# Autodesk Inventor assembly: Catapult Launcher
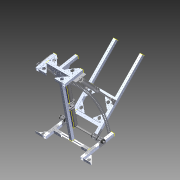
[picture p0: Inventor's stored thumbnail of the model, 180x180]
Saved by Autodesk Inventor 2014 (Build 180170000, 170)
## iProperties
Created: 2014-01-17
Part Number: Catapult Launcher
Document SubType Name: Assembly
Designer: Andrew Toennies
Mass: 5501.43 g
Surface Area: 13469.8 cm^2
Volume: 1150.51 cm^3
Density: 4.78173 g/cm^3
Author: Andrew Toennies
## Documents named in this file (26)
- C:\Users\Michael\Documents\GitHub\2014buildCAD\New Shooter\Catapult Launcher.iam
- C:\Users\Michael\Documents\GitHub\2014buildCAD\New Shooter\Vex Pro 1x1 rectangular tubing 7 in length.ipt
- C:\Users\Michael\Documents\GitHub\2014buildCAD\New Shooter\Vex Pro Side Bearing Gusset - OUT OF STOCK 1192014.ipt
- C:\Users\Michael\Documents\GitHub\2014buildCAD\New Shooter\Vex Pro Corner Gusset - IN STOCK 1192014.ipt
- C:\Users\Michael\Documents\GitHub\2014buildCAD\New Shooter\Bearing ID 0.500 Hex OD 1.125.ipt
- C:\Users\Michael\Documents\GitHub\2014buildCAD\New Shooter\Shaft (Steel 0.500 Hex).ipt
- C:\Users\Michael\Documents\GitHub\2014buildCAD\New Shooter\Vex Pro 1x1 rectangular tubing 27 in length.ipt
- C:\Users\Michael\Documents\GitHub\2014buildCAD\New Shooter\Vex Pro 1x1 rectangular tubing 3 in length.ipt
- C:\Users\Michael\Documents\GitHub\2014buildCAD\New Shooter\Vex Pro 1x1 rectangular tubing 11 in length.ipt
- C:\Users\Michael\Documents\GitHub\2014buildCAD\New Shooter\1.5 in bore 6 in stroke cylinder - BIMBA\176-DP(D-229)(F,D-231-1).iam
- C:\Users\Michael\Documents\GitHub\2014buildCAD\New Shooter\Aluminum Plate (0.125).ipt
- C:\Users\Michael\Documents\GitHub\2014buildCAD\New Shooter\1.5 in bore 6 in stroke cylinder - BIMBA\D-14826.ipt
- C:\Users\Michael\Documents\GitHub\2014buildCAD\New Shooter\1.5 in bore 6 in stroke cylinder - BIMBA\D-9969.ipt
- C:\Users\Michael\Documents\GitHub\2014buildCAD\New Shooter\Vex Pro End Bearing Mount - IN STOCK 1192014.ipt
- C:\Users\Michael\Documents\GitHub\2014buildCAD\New Shooter\Vex Pro 1x1 rectangular tubing 13 in length.ipt
- C:\Users\Michael\Documents\GitHub\2014buildCAD\New Shooter\Vex Pro 1x1 rectangular tubing 25 in length.ipt
- C:\Users\Michael\Documents\GitHub\2014buildCAD\New Shooter\0.5625 in bore 2 in stroke compact cylinder - BIMBA\FO-022.iam
- C:\Users\Michael\Documents\GitHub\2014buildCAD\New Shooter\Vex Pro 1x1 rectangular tubing 8 in length.ipt
- C:\Users\Michael\Documents\GitHub\2014buildCAD\New Shooter\Hex Shaft Collar 1-2 in (7552K500).ipt
- C:\Users\Michael\Documents\GitHub\2014buildCAD\New Shooter\#8 1 in length standoff 93330A459.ipt
- C:\Users\Michael\Documents\GitHub\2014buildCAD\New Shooter\Ramp.ipt
- C:\Users\Michael\Documents\GitHub\2014buildCAD\New folder (2)\Pneumatics_Clippard_AVT-32-16.iam
- C:\Users\Michael\Documents\GitHub\2014buildCAD\New Shooter\Spacer (0.4375 ID whatever OD) aluminum.ipt
- C:\Users\Michael\Documents\GitHub\2014buildCAD\New Shooter\Vex Pro T gusset - OUT OF STOCK 1192014.ipt
- C:\Users\Michael\Documents\GitHub\2014buildCAD\New Shooter\#8 0.250 in length spacer 92510A462.ipt
- C:\Users\Michael\Documents\GitHub\2014buildCAD\New Shooter\#8 0.625 in length spacer 92510A466.ipt
## Components (84 placed, 25 different names)
1. Vex Pro T gusset - OUT OF STOCK 1192014:3 — Mate:388, Flush:73, Flush:74
2. Vex Pro T gusset - OUT OF STOCK 1192014:2 — Mate:376, Flush:71, Flush:72
3. Vex Pro T gusset - OUT OF STOCK 1192014:1 — Mate:375, Flush:69, Flush:70
4. #8 1 in length standoff 93330A459:12 — Mate:342, Mate:343
5. #8 1 in length standoff 93330A459:11 — Mate:340, Mate:341
6. #8 1 in length standoff 93330A459:10 — Mate:338, Mate:339
7. #8 1 in length standoff 93330A459:9 — Mate:336, Mate:337
8. #8 1 in length standoff 93330A459:6 — Mate:325, Mate:326
9. #8 1 in length standoff 93330A459:1 — Mate:319, Mate:320
10. #8 1 in length standoff 93330A459:2 — Mate:321, Mate:322
11. #8 1 in length standoff 93330A459:5 — Mate:323, Mate:324
12. Vex Pro 1x1 rectangular tubing 7 in length:1 — Flush:1, Flush:2, Mate:8, Mate:11, Mate:23, Mate:24, Mate:25, Mate:195, Flush:32, Flush:33, Flush:34, Flush:35, Mate:278, Flush:51, Mate:352, Mate:376, Flush:71, Mate:380, Mate:381
13. Vex Pro 1x1 rectangular tubing 7 in length:2 — Flush:1, Flush:2, Mate:3, Mate:5, Mate:14, Mate:15, Mate:16, Mate:123, Mate:188, Mate:195, Flush:25, Flush:28, Flush:29, Flush:30, Flush:31, Mate:355, Mate:375, Flush:69, Mate:378
14. Vex Pro Side Bearing Gusset - OUT OF STOCK 1192014:1 — Mate:3, Mate:26, Mate:27, Flush:28, Flush:29, Mate:319, Mate:320, Mate:322, Mate:324, Mate:326
15. Vex Pro Side Bearing Gusset - OUT OF STOCK 1192014:2 — Mate:5, Mate:28, Mate:29, Flush:30, Flush:31, Mate:321, Mate:323, Mate:325
16. Vex Pro Side Bearing Gusset - OUT OF STOCK 1192014:3 — Mate:11, Mate:32, Mate:33, Flush:32, Flush:33, Mate:337, Mate:338, Mate:339, Mate:340, Mate:342, Mate:343
17. Vex Pro Side Bearing Gusset - OUT OF STOCK 1192014:4 — Mate:8, Mate:30, Mate:31, Flush:34, Flush:35, Mate:336, Mate:341
18. Vex Pro Corner Gusset - IN STOCK 1192014:2 — Mate:14, Mate:15, Mate:16, Flush:53
19. Vex Pro Corner Gusset - IN STOCK 1192014:4 — Mate:23, Mate:24, Mate:25
20. Bearing ID 0.500 Hex OD 1.125:1 — Mate:28, Mate:29, Flush:3, Flush:5, Mate:306
21. Bearing ID 0.500 Hex OD 1.125:2 — Mate:26, Mate:27, Flush:3, Mate:34, Mate:35, Mate:303
22. Bearing ID 0.500 Hex OD 1.125:3 — Mate:30, Mate:31, Flush:4, Mate:318
23. Bearing ID 0.500 Hex OD 1.125:4 — Mate:32, Mate:33, Flush:4, Flush:5, Mate:69, Mate:315
24. Spacer (0.4375 ID whatever OD) aluminum:1 — Mate:371, Mate:372
25. Spacer (0.4375 ID whatever OD) aluminum:2 — Mate:373, Mate:374
26. Shaft (Steel 0.500 Hex):1 — Mate:34, Mate:35, Flush:25, Mate:227, Mate:228, Mate:301, Mate:302, Mate:304, Mate:305, Mate:307, Mate:308, Mate:310, Mate:311, Mate:313, Mate:314, Mate:316, Mate:317
27. Hex Shaft Collar 1-2 in (7552K500):1 — Mate:301, Mate:302, Mate:303
28. Hex Shaft Collar 1-2 in (7552K500):2 — Mate:307, Mate:308, Mate:309
29. Hex Shaft Collar 1-2 in (7552K500):3 — Mate:304, Mate:305, Mate:306, Mate:371, Mate:372
30. Hex Shaft Collar 1-2 in (7552K500):4 — Mate:310, Mate:311, Mate:312
31. Hex Shaft Collar 1-2 in (7552K500):5 — Mate:313, Mate:314, Mate:315, Mate:373, Mate:374
32. Hex Shaft Collar 1-2 in (7552K500):6 — Mate:316, Mate:317, Mate:318
33. #8 1 in length standoff 93330A459:13 — Mate:350, Mate:351
34. #8 1 in length standoff 93330A459:14 — Mate:348, Mate:349
35. #8 1 in length standoff 93330A459:15 — Mate:346, Mate:347
36. #8 1 in length standoff 93330A459:16 — Mate:344, Mate:345
37. #8 1 in length standoff 93330A459:3 — Mate:327, Mate:328
38. #8 1 in length standoff 93330A459:4 — Mate:329, Mate:330
39. #8 1 in length standoff 93330A459:7 — Mate:334, Mate:335
40. #8 1 in length standoff 93330A459:8 — Mate:332, Mate:333
41. Vex Pro Corner Gusset - IN STOCK 1192014:14 — Mate:250, Mate:251, Flush:45, Mate:271
42. Vex Pro Corner Gusset - IN STOCK 1192014:13 — Mate:252, Mate:253, Flush:46
43. Vex Pro Corner Gusset - IN STOCK 1192014:12 — Mate:248, Mate:249, Flush:44
44. Vex Pro Corner Gusset - IN STOCK 1192014:11 — Mate:243, Flush:43, Mate:244
45. Vex Pro 1x1 rectangular tubing 11 in length:1 — Mate:191, Flush:42, Mate:250, Mate:253, Flush:46, Mate:267
46. Vex Pro 1x1 rectangular tubing 11 in length:2 — Flush:41, Mate:242, Mate:243, Flush:43, Mate:246, Mate:248, Flush:44
47. D-9969:1 — Mate:164, Mate:165, Mate:198, Flush:36, Mate:270, Mate:377
48. D-14826:1 — Mate:164, Mate:169, Mate:170, Flush:37, Mate:247
49. Vex Pro End Bearing Mount - IN STOCK 1192014:4 — Mate:229, Mate:230, Mate:231, Mate:232, Mate:246, Mate:345, Mate:346, Mate:348, Mate:349, Mate:350
50. Vex Pro End Bearing Mount - IN STOCK 1192014:3 — Mate:217, Mate:218, Mate:219, Mate:220, Mate:221, Mate:327, Mate:328, Mate:330, Mate:333, Mate:335
51. Vex Pro End Bearing Mount - IN STOCK 1192014:2 — Mate:233, Mate:234, Mate:235, Mate:236, Mate:245, Mate:344, Mate:347, Mate:351
52. Vex Pro End Bearing Mount - IN STOCK 1192014:1 — Mate:222, Mate:223, Mate:224, Mate:225, Mate:226, Mate:329, Mate:332, Mate:334
53. Vex Pro 1x1 rectangular tubing 27 in length:3 — Mate:198, Mate:229, Mate:230, Mate:231, Mate:233, Mate:234, Mate:235, Flush:27, Flush:36, Flush:41, Mate:242, Mate:244, Mate:251, Flush:45, Mate:267, Mate:270, Mate:271
54. Vex Pro 1x1 rectangular tubing 27 in length:2 — Mate:188, Mate:191, Mate:212, Mate:219, Mate:220, Mate:221, Mate:224, Mate:225, Mate:226, Flush:26, Flush:37, Flush:42, Mate:247, Mate:249, Mate:252
55. Bearing ID 0.500 Hex OD 1.125:5 — Mate:80, Mate:222, Mate:223, Mate:228, Mate:309
56. Bearing ID 0.500 Hex OD 1.125:6 — Mate:80, Mate:217, Mate:218, Mate:227
57. Bearing ID 0.500 Hex OD 1.125:7 — Mate:68, Mate:69, Mate:236, Mate:245
58. Bearing ID 0.500 Hex OD 1.125:8 — Mate:68, Mate:232, Mate:312
59. 176-DP(D-229)(F,D-231-1):1 [sub-assembly] — Mate:153, Mate:154, Mate:155, Mate:165, Mate:171, Mate:377
60. 176-DP(D-229)(F,D-231-1):2 [sub-assembly] — Mate:156, Mate:167, Mate:168, Mate:169, Mate:170, Mate:171
61. Aluminum Plate (0.125):1 — Mate:153, Mate:154, Mate:155, Mate:159, Flush:24
62. Aluminum Plate (0.125):2 — Mate:156, Mate:160, Mate:167, Mate:168, Flush:24, Flush:47
63. Vex Pro 1x1 rectangular tubing 3 in length:2 — Mate:121, Flush:14, Mate:122, Flush:19, Mate:159, Flush:27, Mate:276, Mate:359, Mate:385
64. Vex Pro 1x1 rectangular tubing 3 in length:1 — Flush:13, Mate:118, Mate:119, Mate:120, Mate:123, Flush:19, Mate:160, Mate:212, Flush:26, Flush:47, Mate:272, Flush:48, Mate:273, Mate:275, Mate:360, Mate:387
65. Vex Pro Corner Gusset - IN STOCK 1192014:8 — Flush:13, Mate:118, Mate:119, Mate:120, Flush:17, Flush:53
66. Vex Pro Corner Gusset - IN STOCK 1192014:6 — Mate:121, Flush:14, Mate:122, Flush:17
67. Vex Pro 1x1 rectangular tubing 11 in length:3 — Mate:272, Flush:48, Mate:274, Flush:49, Mate:277, Flush:50, Mate:290, Mate:291, Mate:293, Flush:57, Mate:369, Flush:66
68. Vex Pro Corner Gusset - IN STOCK 1192014:15 — Mate:273, Mate:274, Flush:49, Mate:275
69. Vex Pro Corner Gusset - IN STOCK 1192014:16 — Mate:276, Mate:277, Flush:50
70. Vex Pro 1x1 rectangular tubing 13 in length:1 — Mate:278, Flush:51, Mate:284, Flush:55, Flush:65, Flush:70, Flush:72, Mate:388, Flush:73
71. Vex Pro 1x1 rectangular tubing 25 in length:1 — Mate:284, Flush:55, Mate:285, Mate:287, Mate:288, Mate:289, Flush:56, Mate:292, Mate:300, Flush:63, Mate:367, Flush:64, Mate:368, Flush:67, Flush:74
72. FO-022:1 [sub-assembly] — Mate:285, Mate:287, Mate:288
73. Vex Pro Corner Gusset - IN STOCK 1192014:17 — Mate:289, Mate:290, Flush:56, Mate:291
74. Vex Pro Corner Gusset - IN STOCK 1192014:18 — Mate:292, Mate:293, Flush:57
75. Vex Pro 1x1 rectangular tubing 8 in length:1 — Mate:369, Flush:66, Mate:370, Flush:68
76. Vex Pro Corner Gusset - IN STOCK 1192014:21 — Mate:300, Mate:370, Flush:67, Flush:68
77. #8 0.250 in length spacer 92510A462:1 — Mate:380, Mate:381, Mate:382
78. #8 0.250 in length spacer 92510A462:2 — Mate:378, Mate:379, Mate:383
79. #8 0.625 in length spacer 92510A466:1 — Mate:384, Mate:385
80. #8 0.625 in length spacer 92510A466:2 — Mate:386, Mate:387
81. Ramp:1 — Mate:355, Mate:360, Mate:379, Mate:383, Mate:386
82. Ramp:2 — Mate:352, Mate:359, Mate:382, Mate:384
83. Pneumatics_Clippard_AVT-32-16:1 [sub-assembly] — Flush:63, Mate:367, Flush:65
84. Pneumatics_Clippard_AVT-32-16:2 [sub-assembly] — Flush:64, Mate:368
## Relationships (225: Mate 175, Flush 50)
- Flush:1: Vex Pro 1x1 rectangular tubing 7 in length:1 ↔ Vex Pro 1x1 rectangular tubing 7 in length:2
- Flush:2: Vex Pro 1x1 rectangular tubing 7 in length:1 ↔ Vex Pro 1x1 rectangular tubing 7 in length:2
- Mate:3: Vex Pro 1x1 rectangular tubing 7 in length:2 ↔ Vex Pro Side Bearing Gusset - OUT OF STOCK 1192014:1
- Mate:5: Vex Pro 1x1 rectangular tubing 7 in length:2 ↔ Vex Pro Side Bearing Gusset - OUT OF STOCK 1192014:2
- Mate:8: Vex Pro 1x1 rectangular tubing 7 in length:1 ↔ Vex Pro Side Bearing Gusset - OUT OF STOCK 1192014:4
- Mate:11: Vex Pro 1x1 rectangular tubing 7 in length:1 ↔ Vex Pro Side Bearing Gusset - OUT OF STOCK 1192014:3
- Mate:14: Vex Pro 1x1 rectangular tubing 7 in length:2 ↔ Vex Pro Corner Gusset - IN STOCK 1192014:2
- Mate:15: Vex Pro 1x1 rectangular tubing 7 in length:2 ↔ Vex Pro Corner Gusset - IN STOCK 1192014:2
- Mate:16: Vex Pro 1x1 rectangular tubing 7 in length:2 ↔ Vex Pro Corner Gusset - IN STOCK 1192014:2
- Mate:23: Vex Pro 1x1 rectangular tubing 7 in length:1 ↔ Vex Pro Corner Gusset - IN STOCK 1192014:4
- Mate:24: Vex Pro 1x1 rectangular tubing 7 in length:1 ↔ Vex Pro Corner Gusset - IN STOCK 1192014:4
- Mate:25: Vex Pro 1x1 rectangular tubing 7 in length:1 ↔ Vex Pro Corner Gusset - IN STOCK 1192014:4
- Mate:26: Vex Pro Side Bearing Gusset - OUT OF STOCK 1192014:1 ↔ Bearing ID 0.500 Hex OD 1.125:2
- Mate:27: Vex Pro Side Bearing Gusset - OUT OF STOCK 1192014:1 ↔ Bearing ID 0.500 Hex OD 1.125:2
- Mate:28: Vex Pro Side Bearing Gusset - OUT OF STOCK 1192014:2 ↔ Bearing ID 0.500 Hex OD 1.125:1
- Mate:29: Vex Pro Side Bearing Gusset - OUT OF STOCK 1192014:2 ↔ Bearing ID 0.500 Hex OD 1.125:1
- Flush:3: Bearing ID 0.500 Hex OD 1.125:1 ↔ Bearing ID 0.500 Hex OD 1.125:2
- Mate:30: Vex Pro Side Bearing Gusset - OUT OF STOCK 1192014:4 ↔ Bearing ID 0.500 Hex OD 1.125:3
- Mate:31: Vex Pro Side Bearing Gusset - OUT OF STOCK 1192014:4 ↔ Bearing ID 0.500 Hex OD 1.125:3
- Mate:32: Vex Pro Side Bearing Gusset - OUT OF STOCK 1192014:3 ↔ Bearing ID 0.500 Hex OD 1.125:4
- Mate:33: Vex Pro Side Bearing Gusset - OUT OF STOCK 1192014:3 ↔ Bearing ID 0.500 Hex OD 1.125:4
- Flush:4: Bearing ID 0.500 Hex OD 1.125:3 ↔ Bearing ID 0.500 Hex OD 1.125:4
- Flush:5: Bearing ID 0.500 Hex OD 1.125:1 ↔ Bearing ID 0.500 Hex OD 1.125:4
- Mate:34: Bearing ID 0.500 Hex OD 1.125:2 ↔ Shaft (Steel 0.500 Hex):1
- Mate:35: Bearing ID 0.500 Hex OD 1.125:2 ↔ Shaft (Steel 0.500 Hex):1
- Mate:68: Bearing ID 0.500 Hex OD 1.125:7 ↔ Bearing ID 0.500 Hex OD 1.125:8
- Mate:69: Bearing ID 0.500 Hex OD 1.125:4 ↔ Bearing ID 0.500 Hex OD 1.125:7
- Mate:80: Bearing ID 0.500 Hex OD 1.125:5 ↔ Bearing ID 0.500 Hex OD 1.125:6
- Flush:13: Vex Pro 1x1 rectangular tubing 3 in length:1 ↔ Vex Pro Corner Gusset - IN STOCK 1192014:8
- Mate:118: Vex Pro 1x1 rectangular tubing 3 in length:1 ↔ Vex Pro Corner Gusset - IN STOCK 1192014:8
- Mate:119: Vex Pro 1x1 rectangular tubing 3 in length:1 ↔ Vex Pro Corner Gusset - IN STOCK 1192014:8
- Mate:120: Vex Pro 1x1 rectangular tubing 3 in length:1 ↔ Vex Pro Corner Gusset - IN STOCK 1192014:8
- Mate:121: Vex Pro 1x1 rectangular tubing 3 in length:2 ↔ Vex Pro Corner Gusset - IN STOCK 1192014:6
- Flush:14: Vex Pro 1x1 rectangular tubing 3 in length:2 ↔ Vex Pro Corner Gusset - IN STOCK 1192014:6
- Mate:122: Vex Pro 1x1 rectangular tubing 3 in length:2 ↔ Vex Pro Corner Gusset - IN STOCK 1192014:6
- Flush:17: Vex Pro Corner Gusset - IN STOCK 1192014:8 ↔ Vex Pro Corner Gusset - IN STOCK 1192014:6
- Mate:123 (-685.8 mm): Vex Pro 1x1 rectangular tubing 7 in length:2 ↔ Vex Pro 1x1 rectangular tubing 3 in length:1
- Flush:19: Vex Pro 1x1 rectangular tubing 3 in length:2 ↔ Vex Pro 1x1 rectangular tubing 3 in length:1
- Mate:153: 176-DP(D-229)(F,D-231-1):1 ↔ Aluminum Plate (0.125):1
- Mate:154: 176-DP(D-229)(F,D-231-1):1 ↔ Aluminum Plate (0.125):1
- Mate:155: 176-DP(D-229)(F,D-231-1):1 ↔ Aluminum Plate (0.125):1
- Mate:156: 176-DP(D-229)(F,D-231-1):2 ↔ Aluminum Plate (0.125):2
- Mate:159: Aluminum Plate (0.125):1 ↔ Vex Pro 1x1 rectangular tubing 3 in length:2
- Mate:160: Aluminum Plate (0.125):2 ↔ Vex Pro 1x1 rectangular tubing 3 in length:1
- Mate:164: D-9969:1 ↔ D-14826:1
- Mate:165: D-9969:1 ↔ 176-DP(D-229)(F,D-231-1):1
- Mate:167: 176-DP(D-229)(F,D-231-1):2 ↔ Aluminum Plate (0.125):2
- Mate:168: 176-DP(D-229)(F,D-231-1):2 ↔ Aluminum Plate (0.125):2
- Mate:169: D-14826:1 ↔ 176-DP(D-229)(F,D-231-1):2
- Mate:170: D-14826:1 ↔ 176-DP(D-229)(F,D-231-1):2
- Mate:171: 176-DP(D-229)(F,D-231-1):1 ↔ 176-DP(D-229)(F,D-231-1):2
- Flush:24: Aluminum Plate (0.125):1 ↔ Aluminum Plate (0.125):2
- Mate:188 (25.4 mm): Vex Pro 1x1 rectangular tubing 7 in length:2 ↔ Vex Pro 1x1 rectangular tubing 27 in length:2
- Mate:191: Vex Pro 1x1 rectangular tubing 11 in length:1 ↔ Vex Pro 1x1 rectangular tubing 27 in length:2
- Mate:195 (330.2 mm): Vex Pro 1x1 rectangular tubing 7 in length:1 ↔ Vex Pro 1x1 rectangular tubing 7 in length:2
- Flush:25 (-25.4 mm): Vex Pro 1x1 rectangular tubing 7 in length:2 ↔ Shaft (Steel 0.500 Hex):1
- Mate:198: D-9969:1 ↔ Vex Pro 1x1 rectangular tubing 27 in length:3
- Mate:212: Vex Pro 1x1 rectangular tubing 27 in length:2 ↔ Vex Pro 1x1 rectangular tubing 3 in length:1
- Mate:217: Vex Pro End Bearing Mount - IN STOCK 1192014:3 ↔ Bearing ID 0.500 Hex OD 1.125:6
- Mate:218: Vex Pro End Bearing Mount - IN STOCK 1192014:3 ↔ Bearing ID 0.500 Hex OD 1.125:6
- Mate:219: Vex Pro End Bearing Mount - IN STOCK 1192014:3 ↔ Vex Pro 1x1 rectangular tubing 27 in length:2
- Mate:220: Vex Pro End Bearing Mount - IN STOCK 1192014:3 ↔ Vex Pro 1x1 rectangular tubing 27 in length:2
- Mate:221: Vex Pro End Bearing Mount - IN STOCK 1192014:3 ↔ Vex Pro 1x1 rectangular tubing 27 in length:2
- Mate:222: Vex Pro End Bearing Mount - IN STOCK 1192014:1 ↔ Bearing ID 0.500 Hex OD 1.125:5
- Mate:223: Vex Pro End Bearing Mount - IN STOCK 1192014:1 ↔ Bearing ID 0.500 Hex OD 1.125:5
- Mate:224: Vex Pro End Bearing Mount - IN STOCK 1192014:1 ↔ Vex Pro 1x1 rectangular tubing 27 in length:2
- Mate:225: Vex Pro End Bearing Mount - IN STOCK 1192014:1 ↔ Vex Pro 1x1 rectangular tubing 27 in length:2
- Mate:226: Vex Pro End Bearing Mount - IN STOCK 1192014:1 ↔ Vex Pro 1x1 rectangular tubing 27 in length:2
- Mate:227: Shaft (Steel 0.500 Hex):1 ↔ Bearing ID 0.500 Hex OD 1.125:6
- Mate:228: Shaft (Steel 0.500 Hex):1 ↔ Bearing ID 0.500 Hex OD 1.125:5
- Mate:229: Vex Pro End Bearing Mount - IN STOCK 1192014:4 ↔ Vex Pro 1x1 rectangular tubing 27 in length:3
- Mate:230: Vex Pro End Bearing Mount - IN STOCK 1192014:4 ↔ Vex Pro 1x1 rectangular tubing 27 in length:3
- Mate:231: Vex Pro End Bearing Mount - IN STOCK 1192014:4 ↔ Vex Pro 1x1 rectangular tubing 27 in length:3
- Mate:232: Vex Pro End Bearing Mount - IN STOCK 1192014:4 ↔ Bearing ID 0.500 Hex OD 1.125:8
- Mate:233: Vex Pro End Bearing Mount - IN STOCK 1192014:2 ↔ Vex Pro 1x1 rectangular tubing 27 in length:3
- Mate:234: Vex Pro End Bearing Mount - IN STOCK 1192014:2 ↔ Vex Pro 1x1 rectangular tubing 27 in length:3
- Mate:235: Vex Pro End Bearing Mount - IN STOCK 1192014:2 ↔ Vex Pro 1x1 rectangular tubing 27 in length:3
- Mate:236: Vex Pro End Bearing Mount - IN STOCK 1192014:2 ↔ Bearing ID 0.500 Hex OD 1.125:7
- Flush:26: Vex Pro 1x1 rectangular tubing 27 in length:2 ↔ Vex Pro 1x1 rectangular tubing 3 in length:1
- Flush:27: Vex Pro 1x1 rectangular tubing 27 in length:3 ↔ Vex Pro 1x1 rectangular tubing 3 in length:2
- Flush:28: Vex Pro 1x1 rectangular tubing 7 in length:2 ↔ Vex Pro Side Bearing Gusset - OUT OF STOCK 1192014:1
- Flush:29 (82.55 mm): Vex Pro 1x1 rectangular tubing 7 in length:2 ↔ Vex Pro Side Bearing Gusset - OUT OF STOCK 1192014:1
- Flush:30: Vex Pro 1x1 rectangular tubing 7 in length:2 ↔ Vex Pro Side Bearing Gusset - OUT OF STOCK 1192014:2
- Flush:31 (-82.55 mm): Vex Pro 1x1 rectangular tubing 7 in length:2 ↔ Vex Pro Side Bearing Gusset - OUT OF STOCK 1192014:2
- Flush:32: Vex Pro 1x1 rectangular tubing 7 in length:1 ↔ Vex Pro Side Bearing Gusset - OUT OF STOCK 1192014:3
- Flush:33 (82.55 mm): Vex Pro 1x1 rectangular tubing 7 in length:1 ↔ Vex Pro Side Bearing Gusset - OUT OF STOCK 1192014:3
- Flush:34: Vex Pro 1x1 rectangular tubing 7 in length:1 ↔ Vex Pro Side Bearing Gusset - OUT OF STOCK 1192014:4
- Flush:35 (-82.55 mm): Vex Pro 1x1 rectangular tubing 7 in length:1 ↔ Vex Pro Side Bearing Gusset - OUT OF STOCK 1192014:4
- Flush:36: D-9969:1 ↔ Vex Pro 1x1 rectangular tubing 27 in length:3
- Flush:37: D-14826:1 ↔ Vex Pro 1x1 rectangular tubing 27 in length:2
- Flush:41: Vex Pro 1x1 rectangular tubing 11 in length:2 ↔ Vex Pro 1x1 rectangular tubing 27 in length:3
- Mate:242: Vex Pro 1x1 rectangular tubing 11 in length:2 ↔ Vex Pro 1x1 rectangular tubing 27 in length:3
- Flush:42: Vex Pro 1x1 rectangular tubing 11 in length:1 ↔ Vex Pro 1x1 rectangular tubing 27 in length:2
- Mate:243: Vex Pro Corner Gusset - IN STOCK 1192014:11 ↔ Vex Pro 1x1 rectangular tubing 11 in length:2
- Flush:43: Vex Pro Corner Gusset - IN STOCK 1192014:11 ↔ Vex Pro 1x1 rectangular tubing 11 in length:2
- Mate:244: Vex Pro Corner Gusset - IN STOCK 1192014:11 ↔ Vex Pro 1x1 rectangular tubing 27 in length:3
- Mate:245: Vex Pro End Bearing Mount - IN STOCK 1192014:2 ↔ Bearing ID 0.500 Hex OD 1.125:7
- Mate:246 (6.35 mm): Vex Pro 1x1 rectangular tubing 11 in length:2 ↔ Vex Pro End Bearing Mount - IN STOCK 1192014:4
- Mate:247: D-14826:1 ↔ Vex Pro 1x1 rectangular tubing 27 in length:2
- Mate:248: Vex Pro Corner Gusset - IN STOCK 1192014:12 ↔ Vex Pro 1x1 rectangular tubing 11 in length:2
- Mate:249: Vex Pro Corner Gusset - IN STOCK 1192014:12 ↔ Vex Pro 1x1 rectangular tubing 27 in length:2
- Flush:44: Vex Pro Corner Gusset - IN STOCK 1192014:12 ↔ Vex Pro 1x1 rectangular tubing 11 in length:2
- Mate:250: Vex Pro Corner Gusset - IN STOCK 1192014:14 ↔ Vex Pro 1x1 rectangular tubing 11 in length:1
- Mate:251: Vex Pro Corner Gusset - IN STOCK 1192014:14 ↔ Vex Pro 1x1 rectangular tubing 27 in length:3
- Flush:45: Vex Pro Corner Gusset - IN STOCK 1192014:14 ↔ Vex Pro 1x1 rectangular tubing 27 in length:3
- Mate:252: Vex Pro Corner Gusset - IN STOCK 1192014:13 ↔ Vex Pro 1x1 rectangular tubing 27 in length:2
- Mate:253: Vex Pro Corner Gusset - IN STOCK 1192014:13 ↔ Vex Pro 1x1 rectangular tubing 11 in length:1
- Flush:46: Vex Pro Corner Gusset - IN STOCK 1192014:13 ↔ Vex Pro 1x1 rectangular tubing 11 in length:1
- Mate:267: Vex Pro 1x1 rectangular tubing 11 in length:1 ↔ Vex Pro 1x1 rectangular tubing 27 in length:3
- Flush:47: Aluminum Plate (0.125):2 ↔ Vex Pro 1x1 rectangular tubing 3 in length:1
- Mate:270: D-9969:1 ↔ Vex Pro 1x1 rectangular tubing 27 in length:3
- Mate:271: Vex Pro Corner Gusset - IN STOCK 1192014:14 ↔ Vex Pro 1x1 rectangular tubing 27 in length:3
- Mate:272: Vex Pro 1x1 rectangular tubing 3 in length:1 ↔ Vex Pro 1x1 rectangular tubing 11 in length:3
- Flush:48: Vex Pro 1x1 rectangular tubing 3 in length:1 ↔ Vex Pro 1x1 rectangular tubing 11 in length:3
- Mate:273: Vex Pro 1x1 rectangular tubing 3 in length:1 ↔ Vex Pro Corner Gusset - IN STOCK 1192014:15
- Mate:274: Vex Pro 1x1 rectangular tubing 11 in length:3 ↔ Vex Pro Corner Gusset - IN STOCK 1192014:15
- Flush:49: Vex Pro 1x1 rectangular tubing 11 in length:3 ↔ Vex Pro Corner Gusset - IN STOCK 1192014:15
- Mate:275: Vex Pro 1x1 rectangular tubing 3 in length:1 ↔ Vex Pro Corner Gusset - IN STOCK 1192014:15
- Mate:276: Vex Pro 1x1 rectangular tubing 3 in length:2 ↔ Vex Pro Corner Gusset - IN STOCK 1192014:16
- Mate:277: Vex Pro 1x1 rectangular tubing 11 in length:3 ↔ Vex Pro Corner Gusset - IN STOCK 1192014:16
- Flush:50: Vex Pro 1x1 rectangular tubing 11 in length:3 ↔ Vex Pro Corner Gusset - IN STOCK 1192014:16
- Mate:278: Vex Pro 1x1 rectangular tubing 7 in length:1 ↔ Vex Pro 1x1 rectangular tubing 13 in length:1
- Flush:51: Vex Pro 1x1 rectangular tubing 7 in length:1 ↔ Vex Pro 1x1 rectangular tubing 13 in length:1
- Flush:53: Vex Pro Corner Gusset - IN STOCK 1192014:2 ↔ Vex Pro Corner Gusset - IN STOCK 1192014:8
- Mate:284: Vex Pro 1x1 rectangular tubing 13 in length:1 ↔ Vex Pro 1x1 rectangular tubing 25 in length:1
- Flush:55: Vex Pro 1x1 rectangular tubing 13 in length:1 ↔ Vex Pro 1x1 rectangular tubing 25 in length:1
- Mate:285: Vex Pro 1x1 rectangular tubing 25 in length:1 ↔ FO-022:1
- Mate:287: Vex Pro 1x1 rectangular tubing 25 in length:1 ↔ FO-022:1
- Mate:288: Vex Pro 1x1 rectangular tubing 25 in length:1 ↔ FO-022:1
- Mate:289: Vex Pro 1x1 rectangular tubing 25 in length:1 ↔ Vex Pro Corner Gusset - IN STOCK 1192014:17
- Mate:290: Vex Pro 1x1 rectangular tubing 11 in length:3 ↔ Vex Pro Corner Gusset - IN STOCK 1192014:17
- Flush:56: Vex Pro 1x1 rectangular tubing 25 in length:1 ↔ Vex Pro Corner Gusset - IN STOCK 1192014:17
- Mate:291: Vex Pro 1x1 rectangular tubing 11 in length:3 ↔ Vex Pro Corner Gusset - IN STOCK 1192014:17
- Mate:292: Vex Pro 1x1 rectangular tubing 25 in length:1 ↔ Vex Pro Corner Gusset - IN STOCK 1192014:18
- Mate:293: Vex Pro 1x1 rectangular tubing 11 in length:3 ↔ Vex Pro Corner Gusset - IN STOCK 1192014:18
- Flush:57: Vex Pro 1x1 rectangular tubing 11 in length:3 ↔ Vex Pro Corner Gusset - IN STOCK 1192014:18
- Mate:300: Vex Pro 1x1 rectangular tubing 25 in length:1 ↔ Vex Pro Corner Gusset - IN STOCK 1192014:21
- Mate:301: Shaft (Steel 0.500 Hex):1 ↔ Hex Shaft Collar 1-2 in (7552K500):1
- Mate:302: Shaft (Steel 0.500 Hex):1 ↔ Hex Shaft Collar 1-2 in (7552K500):1
- Mate:303: Bearing ID 0.500 Hex OD 1.125:2 ↔ Hex Shaft Collar 1-2 in (7552K500):1
- Mate:304: Shaft (Steel 0.500 Hex):1 ↔ Hex Shaft Collar 1-2 in (7552K500):3
- Mate:305: Shaft (Steel 0.500 Hex):1 ↔ Hex Shaft Collar 1-2 in (7552K500):3
- Mate:306: Bearing ID 0.500 Hex OD 1.125:1 ↔ Hex Shaft Collar 1-2 in (7552K500):3
- Mate:307: Shaft (Steel 0.500 Hex):1 ↔ Hex Shaft Collar 1-2 in (7552K500):2
- Mate:308: Shaft (Steel 0.500 Hex):1 ↔ Hex Shaft Collar 1-2 in (7552K500):2
- Mate:309: Hex Shaft Collar 1-2 in (7552K500):2 ↔ Bearing ID 0.500 Hex OD 1.125:5
- Mate:310: Shaft (Steel 0.500 Hex):1 ↔ Hex Shaft Collar 1-2 in (7552K500):4
- Mate:311: Shaft (Steel 0.500 Hex):1 ↔ Hex Shaft Collar 1-2 in (7552K500):4
- Mate:312: Hex Shaft Collar 1-2 in (7552K500):4 ↔ Bearing ID 0.500 Hex OD 1.125:8
- Mate:313: Shaft (Steel 0.500 Hex):1 ↔ Hex Shaft Collar 1-2 in (7552K500):5
- Mate:314: Shaft (Steel 0.500 Hex):1 ↔ Hex Shaft Collar 1-2 in (7552K500):5
- Mate:315: Bearing ID 0.500 Hex OD 1.125:4 ↔ Hex Shaft Collar 1-2 in (7552K500):5
- Mate:316: Shaft (Steel 0.500 Hex):1 ↔ Hex Shaft Collar 1-2 in (7552K500):6
- Mate:317: Shaft (Steel 0.500 Hex):1 ↔ Hex Shaft Collar 1-2 in (7552K500):6
- Mate:318: Bearing ID 0.500 Hex OD 1.125:3 ↔ Hex Shaft Collar 1-2 in (7552K500):6
- Mate:319: #8 1 in length standoff 93330A459:1 ↔ Vex Pro Side Bearing Gusset - OUT OF STOCK 1192014:1
- Mate:320: #8 1 in length standoff 93330A459:1 ↔ Vex Pro Side Bearing Gusset - OUT OF STOCK 1192014:1
- Mate:321: #8 1 in length standoff 93330A459:2 ↔ Vex Pro Side Bearing Gusset - OUT OF STOCK 1192014:2
- Mate:322: #8 1 in length standoff 93330A459:2 ↔ Vex Pro Side Bearing Gusset - OUT OF STOCK 1192014:1
- Mate:323: #8 1 in length standoff 93330A459:5 ↔ Vex Pro Side Bearing Gusset - OUT OF STOCK 1192014:2
- Mate:324: #8 1 in length standoff 93330A459:5 ↔ Vex Pro Side Bearing Gusset - OUT OF STOCK 1192014:1
- Mate:325: #8 1 in length standoff 93330A459:6 ↔ Vex Pro Side Bearing Gusset - OUT OF STOCK 1192014:2
- Mate:326: #8 1 in length standoff 93330A459:6 ↔ Vex Pro Side Bearing Gusset - OUT OF STOCK 1192014:1
- Mate:327: #8 1 in length standoff 93330A459:3 ↔ Vex Pro End Bearing Mount - IN STOCK 1192014:3
- Mate:328: #8 1 in length standoff 93330A459:3 ↔ Vex Pro End Bearing Mount - IN STOCK 1192014:3
- Mate:329: #8 1 in length standoff 93330A459:4 ↔ Vex Pro End Bearing Mount - IN STOCK 1192014:1
- Mate:330: #8 1 in length standoff 93330A459:4 ↔ Vex Pro End Bearing Mount - IN STOCK 1192014:3
- Mate:332: #8 1 in length standoff 93330A459:8 ↔ Vex Pro End Bearing Mount - IN STOCK 1192014:1
- Mate:333: #8 1 in length standoff 93330A459:8 ↔ Vex Pro End Bearing Mount - IN STOCK 1192014:3
- Mate:334: #8 1 in length standoff 93330A459:7 ↔ Vex Pro End Bearing Mount - IN STOCK 1192014:1
- Mate:335: #8 1 in length standoff 93330A459:7 ↔ Vex Pro End Bearing Mount - IN STOCK 1192014:3
- Mate:336: #8 1 in length standoff 93330A459:9 ↔ Vex Pro Side Bearing Gusset - OUT OF STOCK 1192014:4
- Mate:337: #8 1 in length standoff 93330A459:9 ↔ Vex Pro Side Bearing Gusset - OUT OF STOCK 1192014:3
- Mate:338: #8 1 in length standoff 93330A459:10 ↔ Vex Pro Side Bearing Gusset - OUT OF STOCK 1192014:3
- Mate:339: #8 1 in length standoff 93330A459:10 ↔ Vex Pro Side Bearing Gusset - OUT OF STOCK 1192014:3
- Mate:340: #8 1 in length standoff 93330A459:11 ↔ Vex Pro Side Bearing Gusset - OUT OF STOCK 1192014:3
- Mate:341: #8 1 in length standoff 93330A459:11 ↔ Vex Pro Side Bearing Gusset - OUT OF STOCK 1192014:4
- Mate:342: #8 1 in length standoff 93330A459:12 ↔ Vex Pro Side Bearing Gusset - OUT OF STOCK 1192014:3
- Mate:343: #8 1 in length standoff 93330A459:12 ↔ Vex Pro Side Bearing Gusset - OUT OF STOCK 1192014:3
- Mate:344: #8 1 in length standoff 93330A459:16 ↔ Vex Pro End Bearing Mount - IN STOCK 1192014:2
- Mate:345: #8 1 in length standoff 93330A459:16 ↔ Vex Pro End Bearing Mount - IN STOCK 1192014:4
- Mate:346: #8 1 in length standoff 93330A459:15 ↔ Vex Pro End Bearing Mount - IN STOCK 1192014:4
- Mate:347: #8 1 in length standoff 93330A459:15 ↔ Vex Pro End Bearing Mount - IN STOCK 1192014:2
- Mate:348: #8 1 in length standoff 93330A459:14 ↔ Vex Pro End Bearing Mount - IN STOCK 1192014:4
- Mate:349: #8 1 in length standoff 93330A459:14 ↔ Vex Pro End Bearing Mount - IN STOCK 1192014:4
- Mate:350: #8 1 in length standoff 93330A459:13 ↔ Vex Pro End Bearing Mount - IN STOCK 1192014:4
- Mate:351: #8 1 in length standoff 93330A459:13 ↔ Vex Pro End Bearing Mount - IN STOCK 1192014:2
- Mate:352: Vex Pro 1x1 rectangular tubing 7 in length:1 ↔ Ramp:2
- Mate:355: Vex Pro 1x1 rectangular tubing 7 in length:2 ↔ Ramp:1
- Mate:359: Vex Pro 1x1 rectangular tubing 3 in length:2 ↔ Ramp:2
- Mate:360: Vex Pro 1x1 rectangular tubing 3 in length:1 ↔ Ramp:1
- Flush:63: Vex Pro 1x1 rectangular tubing 25 in length:1 ↔ Pneumatics_Clippard_AVT-32-16:1
- Mate:367: Vex Pro 1x1 rectangular tubing 25 in length:1 ↔ Pneumatics_Clippard_AVT-32-16:1
- Flush:64: Vex Pro 1x1 rectangular tubing 25 in length:1 ↔ Pneumatics_Clippard_AVT-32-16:2
- Mate:368: Vex Pro 1x1 rectangular tubing 25 in length:1 ↔ Pneumatics_Clippard_AVT-32-16:2
- Flush:65 (127 mm): Vex Pro 1x1 rectangular tubing 13 in length:1 ↔ Pneumatics_Clippard_AVT-32-16:1
- Mate:369: Vex Pro 1x1 rectangular tubing 11 in length:3 ↔ Vex Pro 1x1 rectangular tubing 8 in length:1
- Flush:66: Vex Pro 1x1 rectangular tubing 11 in length:3 ↔ Vex Pro 1x1 rectangular tubing 8 in length:1
- Mate:370: Vex Pro 1x1 rectangular tubing 8 in length:1 ↔ Vex Pro Corner Gusset - IN STOCK 1192014:21
- Flush:67: Vex Pro 1x1 rectangular tubing 25 in length:1 ↔ Vex Pro Corner Gusset - IN STOCK 1192014:21
- Flush:68: Vex Pro 1x1 rectangular tubing 8 in length:1 ↔ Vex Pro Corner Gusset - IN STOCK 1192014:21
- Mate:371: Spacer (0.4375 ID whatever OD) aluminum:1 ↔ Hex Shaft Collar 1-2 in (7552K500):3
- Mate:372: Spacer (0.4375 ID whatever OD) aluminum:1 ↔ Hex Shaft Collar 1-2 in (7552K500):3
- Mate:373: Spacer (0.4375 ID whatever OD) aluminum:2 ↔ Hex Shaft Collar 1-2 in (7552K500):5
- Mate:374: Spacer (0.4375 ID whatever OD) aluminum:2 ↔ Hex Shaft Collar 1-2 in (7552K500):5
- Mate:375: Vex Pro T gusset - OUT OF STOCK 1192014:1 ↔ Vex Pro 1x1 rectangular tubing 7 in length:2
- Flush:69: Vex Pro T gusset - OUT OF STOCK 1192014:1 ↔ Vex Pro 1x1 rectangular tubing 7 in length:2
- Flush:70: Vex Pro T gusset - OUT OF STOCK 1192014:1 ↔ Vex Pro 1x1 rectangular tubing 13 in length:1
- Mate:376: Vex Pro T gusset - OUT OF STOCK 1192014:2 ↔ Vex Pro 1x1 rectangular tubing 7 in length:1
- Flush:71: Vex Pro T gusset - OUT OF STOCK 1192014:2 ↔ Vex Pro 1x1 rectangular tubing 7 in length:1
- Flush:72: Vex Pro T gusset - OUT OF STOCK 1192014:2 ↔ Vex Pro 1x1 rectangular tubing 13 in length:1
- Mate:377: D-9969:1 ↔ 176-DP(D-229)(F,D-231-1):1
- Mate:378: Vex Pro 1x1 rectangular tubing 7 in length:2 ↔ #8 0.250 in length spacer 92510A462:2
- Mate:379: #8 0.250 in length spacer 92510A462:2 ↔ Ramp:1
- Mate:380: Vex Pro 1x1 rectangular tubing 7 in length:1 ↔ #8 0.250 in length spacer 92510A462:1
- Mate:381: Vex Pro 1x1 rectangular tubing 7 in length:1 ↔ #8 0.250 in length spacer 92510A462:1
- Mate:382: #8 0.250 in length spacer 92510A462:1 ↔ Ramp:2
- Mate:383: #8 0.250 in length spacer 92510A462:2 ↔ Ramp:1
- Mate:384: #8 0.625 in length spacer 92510A466:1 ↔ Ramp:2
- Mate:385: Vex Pro 1x1 rectangular tubing 3 in length:2 ↔ #8 0.625 in length spacer 92510A466:1
- Mate:386: #8 0.625 in length spacer 92510A466:2 ↔ Ramp:1
- Mate:387: Vex Pro 1x1 rectangular tubing 3 in length:1 ↔ #8 0.625 in length spacer 92510A466:2
- Mate:388: Vex Pro T gusset - OUT OF STOCK 1192014:3 ↔ Vex Pro 1x1 rectangular tubing 13 in length:1
- Flush:73: Vex Pro T gusset - OUT OF STOCK 1192014:3 ↔ Vex Pro 1x1 rectangular tubing 13 in length:1
- Flush:74: Vex Pro T gusset - OUT OF STOCK 1192014:3 ↔ Vex Pro 1x1 rectangular tubing 25 in length:1
